# Autodesk Inventor assembly: v.2
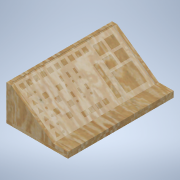
[picture p0: Inventor's stored thumbnail of the model, 180x180]
Saved by Autodesk Inventor 2021 (Build 250183000, 183)
## iProperties
Created: 2020-07-16
Part Number: v.2
Document SubType Name: Assembly
Designer: adick
Author: adick
## Documents named in this file (7)
- C:\Users\adick\Documents\Inventor CAD\Kerbal Kontroller\v.2.iam
- C:\Users\adick\Documents\Inventor CAD\Kerbal Kontroller\Bottom.ipt
- C:\Users\adick\Documents\Inventor CAD\Kerbal Kontroller\Side.ipt
- C:\Users\adick\Documents\Inventor CAD\Kerbal Kontroller\Back.ipt
- C:\Users\adick\Documents\Inventor CAD\Kerbal Kontroller\Front.ipt
- C:\Users\adick\Documents\Inventor CAD\Plexi.ipt
- C:\Users\adick\Documents\Inventor CAD\Kerbal Kontroller\Backplane.ipt
## Components (7 placed, 6 different names)
1. Bottom:1 — Flush:1, Mate:1, Mate:2, Mate:3, Mate:4, Mate:7
2. Side:1 — Flush:1, Mate:3, Mate:4, Mate:5
3. Side:2 — Mate:1, Mate:2, Flush:2, Flush:3, Mate:6, Flush:4
4. Back:1 — Flush:2
5. Front:1 — Flush:3, Mate:7, Mate:8
6. Plexi:1 — Mate:5, Mate:6, Mate:8
7. Backplane:1 — Flush:4
## Relationships (12: Mate 8, Flush 4)
- Flush:1: Bottom:1 ↔ Side:1
- Mate:1: Bottom:1 ↔ Side:2
- Mate:2: Bottom:1 ↔ Side:2
- Mate:3: Bottom:1 ↔ Side:1
- Mate:4: Bottom:1 ↔ Side:1
- Flush:2: Side:2 ↔ Back:1
- Flush:3: Side:2 ↔ Front:1
- Mate:5: Side:1 ↔ Plexi:1
- Mate:6: Side:2 ↔ Plexi:1
- Mate:7: Bottom:1 ↔ Front:1
- Mate:8: Front:1 ↔ Plexi:1
- Flush:4: Side:2 ↔ Backplane:1
